# Autodesk Inventor assembly: Robot A
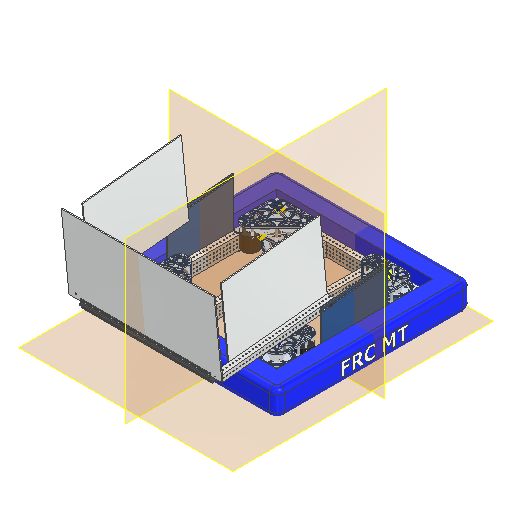
[picture p0: Inventor's stored thumbnail of the model, 512x512]
Saved by Autodesk Inventor 2025.3 (Build 293356000, 356)
## iProperties
Created: 2026-05-20
Part Number: Robot A
Document SubType Name: Assembly
Designer: djair.oliveira
Author: djair.oliveira
## Documents named in this file (4)
- C:\Users\djair.oliveira\Documents\GitHub\MT_2026\CAD\Model A\Robot A.iam
- C:\Users\djair.oliveira\Documents\GitHub\MT_2026\CAD\Model A\Chassi\Chassi.iam
- C:\Users\djair.oliveira\Documents\GitHub\MT_2026\CAD\Model A\Intake\Intake.iam
- C:\Users\djair.oliveira\Documents\GitHub\MT_2026\CAD\Model A\Bumper.ipt
## Components (3 placed, 3 different names)
1. Chassi:1 [sub-assembly] — Alinhado:1, Alinhado:2, Alinhado:3, Coincidente:1, Coincidente:2, Coincidente:3, Coincidente:5
2. Intake:1 [sub-assembly] — Coincidente:1, Coincidente:2, Coincidente:3, Coincidente:4
3. Bumper:1 — Coincidente:4, Coincidente:5
## Relationships (8: Mate 5, Flush 3)
- Alinhado:1 [Flush]: Chassi:1
- Alinhado:2 [Flush]: Chassi:1
- Alinhado:3 [Flush]: Chassi:1
- Coincidente:1 [Mate]: Chassi:1 ↔ Intake:1
- Coincidente:2 [Mate]: Chassi:1 ↔ Intake:1
- Coincidente:3 [Mate]: Chassi:1 ↔ Intake:1
- Coincidente:4 [Mate] (1 mm): Intake:1 ↔ Bumper:1
- Coincidente:5 [Mate] (5 mm): Chassi:1 ↔ Bumper:1
